# Autodesk Inventor assembly: motor_plus_encoder
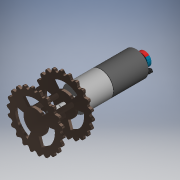
[picture p0: Inventor's stored thumbnail of the model, 180x180]
Saved by Autodesk Inventor 2019.4 (Build 234330000, 330)
## iProperties
Part Number: motor_plus_encoder
Document SubType Name: Assembly
Designer: Jorge
Author: Jorge
## Documents named in this file (3)
- D:\TFG\dev\hardware\ROVER\motor_plus_encoder.iam
- D:\TFG\dev\hardware\ROVER\platform_sprocket.ipt
- D:\TFG\dev\hardware\ROVER\motor.iam
## Components (2 placed, 2 different names)
1. platform_sprocket:1 — Mate:1, Mate:2
2. motor:1 [sub-assembly] — Mate:1, Mate:2
## Relationships (2: Mate 2)
- Mate:1: platform_sprocket:1 ↔ motor:1
- Mate:2 (15 mm): platform_sprocket:1 ↔ motor:1
